# Autodesk Inventor assembly: Drive V2
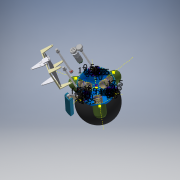
[picture p0: Inventor's stored thumbnail of the model, 180x180]
Saved by Autodesk Inventor 2019.1 (Build 231200000, 200)
## iProperties
Created: 2018-06-30
Part Number: Drive V2
Material: Generisch
Document SubType Name: Assembly
Designer: JochenAlt
Author: JochenAlt
## Documents named in this file (10)
- D:\Projects\Ondine\CAD\Drive V2.iam
- D:\Projects\Ondine\CAD\Sphere.ipt
- D:\Projects\Ondine\CAD\Spindle\SpindleWithGear.ipt
- D:\Projects\Ondine\CAD\Spindle\Spindle.ipt
- D:\Projects\Ondine\CAD\Bearings\W 61700 X-2RS1.iam
- D:\Projects\Ondine\CAD\SpindleMotor.iam
- D:\Projects\Ondine\CAD\PCB\ControllerPCBHolder.ipt
- D:\Projects\Ondine\CAD\PCB\MotorController.ipt
- D:\Projects\Ondine\CAD\Leg\Leg.iam
- D:\Projects\Ondine\CAD\DriveChainEnclosure V2.ipt
## Components (18 placed, 8 different names)
1. Sphere:1 — Passend:38, Passend:127, Passend:129
2. Spindle:1 — Passend:66, Passend:72, Passend:77, Fluchtend:1
3. Spindle:2 — Passend:67, Passend:75, Passend:76
4. Spindle:3 — Passend:73, Passend:114, Passend:117
5. W 61700 X-2RS1:1 [sub-assembly] — Passend:66
6. W 61700 X-2RS1:2 [sub-assembly]
7. W 61700 X-2RS1:3 [sub-assembly] — Passend:67
8. W 61700 X-2RS1:4 [sub-assembly] — Passend:72, Passend:77
9. W 61700 X-2RS1:5 [sub-assembly] — Passend:75, Passend:76
10. W 61700 X-2RS1:6 [sub-assembly] — Passend:73, Passend:117
11. SpindleMotor:1 [sub-assembly] — Fluchtend:1
12. PCBHolder:1 — Passend:125, Passend:126
13. MotorController:1 — Passend:125, Passend:126
14. W 61700 X-2RS1:7 [sub-assembly] — Passend:114
15. Leg:1 [sub-assembly] — Winkel:1, Passend:136, Passend:137, Passend:138
16. DriveChainEnclosure:1 — Passend:129, Passend:130, Passend:131, Passend:133, Passend:134
17. DriveChainEnclosure:2 — Passend:130, Passend:134, Passend:135
18. DriveChainEnclosure:3 — Passend:127, Passend:131, Passend:133, Passend:135, Winkel:1, Passend:136, Passend:137, Passend:138
## Relationships (24: Mate 22, Flush 1, Angle 1)
- Passend:38 [Mate]: Sphere:1
- Passend:66 [Mate]: Spindle:1 ↔ W 61700 X-2RS1:1
- Passend:67 [Mate]: Spindle:2 ↔ W 61700 X-2RS1:3
- Passend:72 [Mate]: Spindle:1 ↔ W 61700 X-2RS1:4
- Passend:73 [Mate]: Spindle:3 ↔ W 61700 X-2RS1:6
- Passend:75 [Mate]: Spindle:2 ↔ W 61700 X-2RS1:5
- Passend:76 [Mate]: Spindle:2 ↔ W 61700 X-2RS1:5
- Passend:77 [Mate]: Spindle:1 ↔ W 61700 X-2RS1:4
- Fluchtend:1 [Flush]: Spindle:1 ↔ SpindleMotor:1
- Passend:114 [Mate]: Spindle:3 ↔ W 61700 X-2RS1:7
- Passend:117 [Mate]: Spindle:3 ↔ W 61700 X-2RS1:6
- Passend:125 [Mate]: PCBHolder:1 ↔ MotorController:1
- Passend:126 [Mate]: PCBHolder:1 ↔ MotorController:1
- Passend:127 [Mate]: Sphere:1 ↔ DriveChainEnclosure:3
- Passend:129 [Mate]: Sphere:1 ↔ DriveChainEnclosure:1
- Passend:130 [Mate]: DriveChainEnclosure:1 ↔ DriveChainEnclosure:2
- Passend:131 [Mate]: DriveChainEnclosure:1 ↔ DriveChainEnclosure:3
- Passend:133 [Mate]: DriveChainEnclosure:1 ↔ DriveChainEnclosure:3
- Passend:134 [Mate]: DriveChainEnclosure:1 ↔ DriveChainEnclosure:2
- Passend:135 [Mate]: DriveChainEnclosure:2 ↔ DriveChainEnclosure:3
- Winkel:1 [Angle] (0 deg): Leg:1 ↔ DriveChainEnclosure:3
- Passend:136 [Mate] (0.2 mm): Leg:1 ↔ DriveChainEnclosure:3
- Passend:137 [Mate] (0.2 mm): Leg:1 ↔ DriveChainEnclosure:3
- Passend:138 [Mate] (0.2 mm): Leg:1 ↔ DriveChainEnclosure:3
